# Autodesk Inventor assembly: TomatoArm1
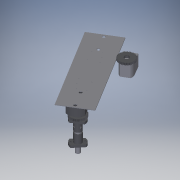
[picture p0: Inventor's stored thumbnail of the model, 180x180]
Saved by Autodesk Inventor 2016 (Build 200138000, 138)
## iProperties
Created: 2016-06-28
Part Number: TomatoArm1
Material: 一般
Document SubType Name: Assembly
Designer: 宏太
Author: 宏太
## Documents named in this file (10)
- C:\Users\宏太\Documents\GitHub\Tomato2016\TomatoArm1.iam
- C:\Users\宏太\Documents\Inventor\Content Center Files\Tomoto2016\NFS5-2020-260.ipt
- C:\Users\宏太\Documents\GitHub\Tomato2016\bottom_board.ipt
- C:\Users\宏太\Documents\GitHub\Tomato2016\shaft2016.ipt
- C:\Users\宏太\Documents\GitHub\Tomato2016\GEAHBB1.0-40-6-A-12\GEAHBB1_0-40-6-A-12.iam
- C:\Users\宏太\Documents\GitHub\Tomato2016\GEAHBB1.0-40-6-B-12\GEAHBB1_0-40-6-B-12.iam
- C:\Users\宏太\Documents\GitHub\Tomato2016\STHCBT15-MB.iam
- C:\Users\宏太\Documents\GitHub\Tomato2016\Servo.iam
- C:\Users\宏太\Documents\Inventor\Content Center Files\Tomoto2016\Side_board.ipt
- C:\Users\宏太\Documents\GitHub\Tomato2016\BGCSB12\BGCSB12.iam
## Components (24 placed, 9 different names)
1. NFS5-2020-260:2 — フラッシュ:12, フラッシュ:13, メイト:6
2. NFS5-2020-260:4 — フラッシュ:10, フラッシュ:11
3. NFS5-2020-260:5 — フラッシュ:17, メイト:7, フラッシュ:18, メイト:11
4. NFS5-2020-260:6 — フラッシュ:14, フラッシュ:15, フラッシュ:16, メイト:13
5. bottom_board:1 — フラッシュ:9, フラッシュ:10, フラッシュ:11, フラッシュ:12, フラッシュ:13, メイト:6, メイト:12
6. shaft2016:1 — 挿入:15, 挿入:16, 挿入:21
7. shaft2016:2 — 挿入:17, 挿入:18, 挿入:22, 挿入:31
8. GEAHBB1_0-40-6-A-12:1 [sub-assembly] — 挿入:26
9. GEAHBB1_0-40-6-A-12:2 [sub-assembly] — 挿入:27
10. GEAHBB1_0-40-6-B-12:1 [sub-assembly] — 挿入:22
11. GEAHBB1_0-40-6-B-12:2 [sub-assembly] — 挿入:21
12. bottom_board:2 — フラッシュ:14, フラッシュ:15, フラッシュ:16, フラッシュ:17, メイト:7, フラッシュ:18, メイト:10, フラッシュ:23, フラッシュ:24, 挿入:28, 挿入:29, 挿入:30
13. STHCBT15-MB:1 [sub-assembly] — 挿入:16
14. STHCBT15-MB:2 [sub-assembly] — 挿入:18
15. STHCBT15-MB:3 [sub-assembly] — 挿入:17
16. STHCBT15-MB:4 [sub-assembly] — 挿入:15
17. Servo:1 [sub-assembly] — 挿入:26
18. Servo:2 [sub-assembly] — 挿入:27, 挿入:28
19. Side_board:1 — メイト:10, フラッシュ:23, メイト:11
20. Side_board:2 — フラッシュ:24, メイト:12, メイト:13
21. BGCSB12:1 [sub-assembly]
22. BGCSB12:2 [sub-assembly]
23. BGCSB12:3 [sub-assembly]
24. BGCSB12:4 [sub-assembly] — 挿入:29, 挿入:30, 挿入:31
## Relationships (30: Flush 12, Insert 12, Mate 6)
- フラッシュ:9 [Flush]: bottom_board:1
- フラッシュ:10 [Flush]: NFS5-2020-260:4 ↔ bottom_board:1
- フラッシュ:11 [Flush]: NFS5-2020-260:4 ↔ bottom_board:1
- フラッシュ:12 [Flush]: NFS5-2020-260:2 ↔ bottom_board:1
- フラッシュ:13 [Flush]: NFS5-2020-260:2 ↔ bottom_board:1
- メイト:6 [Mate]: NFS5-2020-260:2 ↔ bottom_board:1
- 挿入:15 [Insert] (60 mm): shaft2016:1 ↔ STHCBT15-MB:4
- 挿入:16 [Insert] (-55 mm): shaft2016:1 ↔ STHCBT15-MB:1
- 挿入:17 [Insert] (60 mm): shaft2016:2 ↔ STHCBT15-MB:3
- 挿入:18 [Insert] (-55 mm): shaft2016:2 ↔ STHCBT15-MB:2
- 挿入:21 [Insert] (-20 mm): shaft2016:1 ↔ GEAHBB1_0-40-6-B-12:2
- 挿入:22 [Insert] (-20 mm): shaft2016:2 ↔ GEAHBB1_0-40-6-B-12:1
- フラッシュ:14 [Flush]: NFS5-2020-260:6 ↔ bottom_board:2
- フラッシュ:15 [Flush]: NFS5-2020-260:6 ↔ bottom_board:2
- フラッシュ:16 [Flush] (2 mm): NFS5-2020-260:6 ↔ bottom_board:2
- フラッシュ:17 [Flush]: NFS5-2020-260:5 ↔ bottom_board:2
- メイト:7 [Mate]: NFS5-2020-260:5 ↔ bottom_board:2
- フラッシュ:18 [Flush]: NFS5-2020-260:5 ↔ bottom_board:2
- 挿入:26 [Insert]: GEAHBB1_0-40-6-A-12:1 ↔ Servo:1
- 挿入:27 [Insert]: GEAHBB1_0-40-6-A-12:2 ↔ Servo:2
- メイト:10 [Mate]: bottom_board:2 ↔ Side_board:1
- フラッシュ:23 [Flush] (60 mm): bottom_board:2 ↔ Side_board:1
- メイト:11 [Mate]: NFS5-2020-260:5 ↔ Side_board:1
- フラッシュ:24 [Flush] (60 mm): bottom_board:2 ↔ Side_board:2
- メイト:12 [Mate]: bottom_board:1 ↔ Side_board:2
- メイト:13 [Mate]: NFS5-2020-260:6 ↔ Side_board:2
- 挿入:28 [Insert]: bottom_board:2 ↔ Servo:2
- 挿入:29 [Insert]: bottom_board:2 ↔ BGCSB12:4
- 挿入:30 [Insert]: bottom_board:2 ↔ BGCSB12:4
- 挿入:31 [Insert]: shaft2016:2 ↔ BGCSB12:4
